# Autodesk Inventor assembly: Assembly2
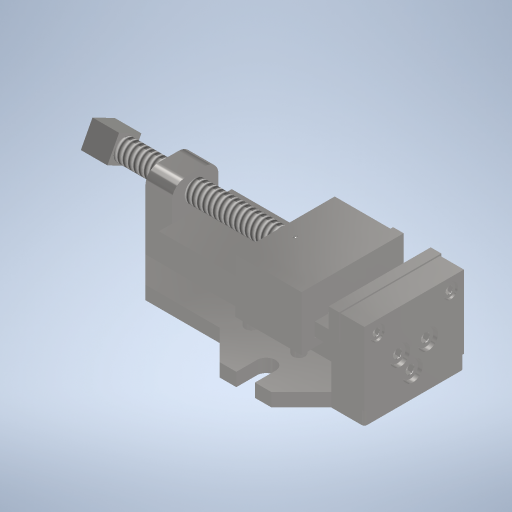
[picture p0: Inventor's stored thumbnail of the model, 512x512]
Saved by Autodesk Inventor 2023.2 (Build 272271000, 271)
## iProperties
Created: 2023-02-07
Part Number: Assembly2
Document SubType Name: Assembly
Designer: manas
Author: manas
## Documents named in this file (17)
- D:\Inventor Files\Assembly2\Assembly2.iam
- D:\Inventor Files\Assembly2\Grundplate.ipt
- D:\Inventor Files\Assembly2\Fuehrung.ipt
- D:\Inventor Files\Assembly2\Feste backe.ipt
- D:\Inventor Files\Assembly2\lose back.ipt
- D:\Inventor Files\Assembly2\Spindel scokel.ipt
- D:\Inventor Files\Assembly2\spindel.ipt
- D:\Inventor Files\Assembly2\druckhuelse.ipt
- D:\Inventor Files\Assembly2\Funrungesch.ipt
- D:\Inventor Files\Assembly2\Spann backe.ipt
- D:\Inventor Files\Assembly2\M 8x35.ipt
- C:\Users\manas\Documents\Inventor\Content Center Files\R2023\en-US\M\M 6x40.ipt
- C:\Users\manas\Documents\Inventor\Content Center Files\R2023\en-US\M\M 6x25.ipt
- C:\Users\manas\Documents\Inventor\Content Center Files\R2023\en-US\M\M 6x16.ipt
- C:\Users\manas\Documents\Inventor\Content Center Files\R2023\en-US\M\M 6x10.ipt
- C:\Users\manas\Documents\Inventor\Content Center Files\R2023\en-US\DIN 916\DIN 916 - M3  x  10.ipt
- C:\Users\manas\Documents\Inventor\Content Center Files\R2023\en-US\M\M 5x16.ipt
## Components (33 placed, 16 different names)
1. Grundplate:1 — Mate:1, Mate:2, Mate:3, Mate:4, Mate:5, Mate:6, Mate:7, Mate:8, Mate:14, Insert:14, Insert:15, Insert:16, Insert:17, Insert:18, Insert:19
2. Fuehrung:1 — Mate:1, Mate:2, Mate:3, Mate:4, Mate:5, Mate:6, Mate:7, Mate:9, Mate:10, Mate:11, Mate:12, Mate:13, Mate:15, Mate:16, Mate:17, Mate:18, Mate:31, Mate:32
3. Feste backe:1 — Mate:14, Mate:15, Mate:16, Mate:17, Mate:18, Mate:19, Mate:20, Mate:21, Insert:3, Insert:4, Insert:5, Insert:12, Insert:13
4. lose back:1 — Mate:22, Mate:23, Mate:24, Mate:25, Mate:26, Mate:27, Mate:28, Mate:29, Mate:30, Mate:31, Mate:32, Insert:1, Insert:6, Insert:7, Mate:33, Insert:20
5. Spindel scokel:1 — Mate:8, Mate:9, Mate:10, Mate:11, Mate:12, Mate:13, Insert:8, Insert:9, Insert:10, Insert:11
6. spindel:1 — Insert:2
7. druckhuelse:1 — Insert:1, Insert:2
8. Funrungesch:1 — Mate:28, Mate:29, Mate:30, Insert:23, Insert:24
9. Funrungesch:2 — Mate:25, Mate:26, Mate:27, Insert:21, Insert:22
10. Spann backe:1 — Mate:22, Mate:23, Mate:24
11. Spann backe:2 — Mate:19, Mate:20, Mate:21
12. M 8x35:2 — Insert:3
13. M 8x35:3 — Insert:4
14. M 8x35:4 — Insert:5
15. M 6x40:1 — Insert:7
16. M 6x40:2 — Insert:6
17. M 6x25:1 — Insert:10
18. M 6x25:2 — Insert:8
19. M 6x25:3 — Insert:9
20. M 6x25:4 — Insert:11
21. M 6x16:1 — Insert:13
22. M 6x16:2 — Insert:12
23. M 6x10:1 — Insert:19
24. M 6x10:2 — Insert:17
25. M 6x10:3 — Insert:18
26. M 6x10:4 — Insert:16
27. M 6x10:5 — Insert:15
28. M 6x10:6 — Insert:14
29. DIN 916 M3  x  10:1 — Mate:33, Insert:20
30. M 5x16:1 — Insert:22
31. M 5x16:2 — Insert:21
32. M 5x16:3 — Insert:24
33. M 5x16:4 — Insert:23
## Relationships (57: Mate 33, Insert 24)
- Mate:1: Grundplate:1 ↔ Fuehrung:1
- Mate:2: Grundplate:1 ↔ Fuehrung:1
- Mate:3: Grundplate:1 ↔ Fuehrung:1
- Mate:4: Grundplate:1 ↔ Fuehrung:1
- Mate:5: Grundplate:1 ↔ Fuehrung:1
- Mate:6: Grundplate:1 ↔ Fuehrung:1
- Mate:7: Grundplate:1 ↔ Fuehrung:1
- Mate:8: Grundplate:1 ↔ Spindel scokel:1
- Mate:9: Fuehrung:1 ↔ Spindel scokel:1
- Mate:10: Fuehrung:1 ↔ Spindel scokel:1
- Mate:11: Fuehrung:1 ↔ Spindel scokel:1
- Mate:12: Fuehrung:1 ↔ Spindel scokel:1
- Mate:13: Fuehrung:1 ↔ Spindel scokel:1
- Mate:14: Grundplate:1 ↔ Feste backe:1
- Mate:15: Fuehrung:1 ↔ Feste backe:1
- Mate:16: Fuehrung:1 ↔ Feste backe:1
- Mate:17: Fuehrung:1 ↔ Feste backe:1
- Mate:18: Fuehrung:1 ↔ Feste backe:1
- Mate:19: Feste backe:1 ↔ Spann backe:2
- Mate:20: Feste backe:1 ↔ Spann backe:2
- Mate:21: Feste backe:1 ↔ Spann backe:2
- Mate:22: lose back:1 ↔ Spann backe:1
- Mate:23: lose back:1 ↔ Spann backe:1
- Mate:24: lose back:1 ↔ Spann backe:1
- Mate:25: lose back:1 ↔ Funrungesch:2
- Mate:26: lose back:1 ↔ Funrungesch:2
- Mate:27: lose back:1 ↔ Funrungesch:2
- Mate:28: lose back:1 ↔ Funrungesch:1
- Mate:29: lose back:1 ↔ Funrungesch:1
- Mate:30: lose back:1 ↔ Funrungesch:1
- Mate:31: Fuehrung:1 ↔ lose back:1
- Mate:32: Fuehrung:1 ↔ lose back:1
- Insert:1: lose back:1 ↔ druckhuelse:1
- Insert:2: spindel:1 ↔ druckhuelse:1
- Insert:3: Feste backe:1 ↔ M 8x35:2
- Insert:4: Feste backe:1 ↔ M 8x35:3
- Insert:5: Feste backe:1 ↔ M 8x35:4
- Insert:6: lose back:1 ↔ M 6x40:2
- Insert:7: lose back:1 ↔ M 6x40:1
- Insert:8: Spindel scokel:1 ↔ M 6x25:2
- Insert:9: Spindel scokel:1 ↔ M 6x25:3
- Insert:10: Spindel scokel:1 ↔ M 6x25:1
- Insert:11: Spindel scokel:1 ↔ M 6x25:4
- Insert:12: Feste backe:1 ↔ M 6x16:2
- Insert:13: Feste backe:1 ↔ M 6x16:1
- Insert:14: Grundplate:1 ↔ M 6x10:6
- Insert:15: Grundplate:1 ↔ M 6x10:5
- Insert:16: Grundplate:1 ↔ M 6x10:4
- Insert:17: Grundplate:1 ↔ M 6x10:2
- Insert:18: Grundplate:1 ↔ M 6x10:3
- Insert:19: Grundplate:1 ↔ M 6x10:1
- Mate:33: lose back:1 ↔ DIN 916 M3  x  10:1
- Insert:20: lose back:1 ↔ DIN 916 M3  x  10:1
- Insert:21: Funrungesch:2 ↔ M 5x16:2
- Insert:22: Funrungesch:2 ↔ M 5x16:1
- Insert:23: Funrungesch:1 ↔ M 5x16:4
- Insert:24: Funrungesch:1 ↔ M 5x16:3
